# Autodesk Inventor assembly: Zonnepaneel 3.0
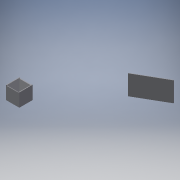
[picture p0: Inventor's stored thumbnail of the model, 180x180]
Saved by Autodesk Inventor 2018.3 (Build 223284000, 284)
## iProperties
Created: 2020-11-19
Part Number: Zonnepaneel 3.0
Document SubType Name: Assembly
Designer: daanv
Author: daanv
## Documents named in this file (8)
- C:\Users\daanv\OneDrive\Documenten\Life\Avans Project RED\Token\Zonnepaneel\V3.0\Zonnepaneel 3.0.iam
- C:\Users\daanv\OneDrive\Documenten\Life\Avans Project RED\Token\Zonnepaneel\V3.0\Bovenplaat.ipt
- C:\Users\daanv\OneDrive\Documenten\Life\Avans Project RED\Token\Zonnepaneel\V3.0\Grondplaat.ipt
- C:\Users\daanv\OneDrive\Documenten\Life\Avans Project RED\Token\Zonnepaneel\V3.0\Zijplaat 1.ipt
- C:\Users\daanv\OneDrive\Documenten\Life\Avans Project RED\Token\Zonnepaneel\V3.0\Zijplaat 2.ipt
- C:\Users\daanv\OneDrive\Documenten\Life\Avans Project RED\Token\Zonnepaneel\V3.0\Zijplaat 3.ipt
- C:\Users\daanv\OneDrive\Documenten\Life\Avans Project RED\Token\Zonnepaneel\V3.0\Zijplaat 4.ipt
- C:\Users\daanv\OneDrive\Documenten\Life\Avans Project RED\Token\Zonnepaneel\V3.0\Zonnecel.ipt
## Components (7 placed, 7 different names)
1. Bovenplaat:1 — Mate:10, Mate:11, Mate:12
2. Grondplaat:1 — Mate:1, Mate:2, Mate:3, Mate:4, Mate:6, Mate:8
3. Zijplaat 1:1 — Mate:1, Mate:2, Mate:7, Mate:11
4. Zijplaat 2:1 — Mate:3, Mate:4, Mate:9, Mate:10
5. Zijplaat 3:1 — Mate:6, Mate:7, Mate:12
6. Zijplaat 4:1 — Mate:8, Mate:9
7. Zonnecel:1
## Relationships (11: Mate 11)
- Mate:1: Grondplaat:1 ↔ Zijplaat 1:1
- Mate:2: Grondplaat:1 ↔ Zijplaat 1:1
- Mate:3: Grondplaat:1 ↔ Zijplaat 2:1
- Mate:4: Grondplaat:1 ↔ Zijplaat 2:1
- Mate:6: Grondplaat:1 ↔ Zijplaat 3:1
- Mate:7: Zijplaat 1:1 ↔ Zijplaat 3:1
- Mate:8: Grondplaat:1 ↔ Zijplaat 4:1
- Mate:9: Zijplaat 2:1 ↔ Zijplaat 4:1
- Mate:10: Bovenplaat:1 ↔ Zijplaat 2:1
- Mate:11: Bovenplaat:1 ↔ Zijplaat 1:1
- Mate:12: Bovenplaat:1 ↔ Zijplaat 3:1
